# Autodesk Inventor assembly: Pipette Assembly
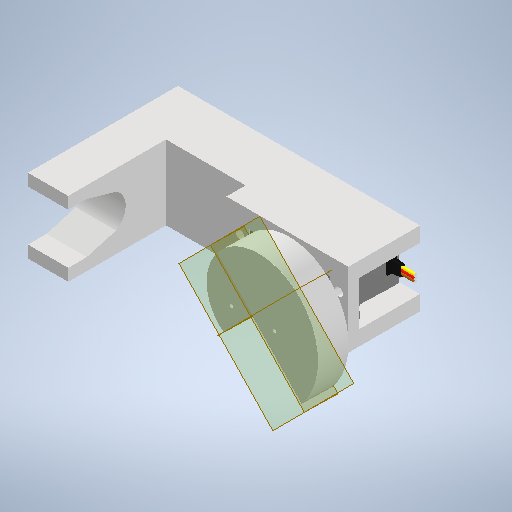
[picture p0: Inventor's stored thumbnail of the model, 512x512]
Saved by Autodesk Inventor 2025.1 (Build 291241000, 241)
## iProperties
Created: 2024-10-19
Part Number: Pipette Assembly
Document SubType Name: Assembly
Designer: 13156
Author: 13156
## Documents named in this file (5)
- C:\Users\13156\Documents\GitHub\Perovskite-Automated-Synthesis-System\CAD\Pipette Assembly.iam
- C:\Users\13156\Downloads\mg996r-servo-3.snapshot.9\mg996R_v2\mg996R_v2\mg996R_v2.ipt
- C:\Users\13156\Desktop\Servo CAD\mg996_arm_2pad\mg996_arm_2pad\mg996_arm_2pad.ipt
- C:\Users\13156\Documents\GitHub\Perovskite-Automated-Synthesis-System\CAD\Holder2.ipt
- C:\Users\13156\Documents\GitHub\Perovskite-Automated-Synthesis-System\CAD\Cam.ipt
## Components (4 placed, 4 different names)
1. mg996R_v2:1 — Mate:1, Insert:1
2. mg996_arm_2pad:1 — Mate:1, Insert:1
3. Holder2:1
4. Cam:1
## Relationships (2: Mate 1, Insert 1)
- Mate:1 (1.5 mm): mg996R_v2:1 ↔ mg996_arm_2pad:1
- Insert:1: mg996R_v2:1 ↔ mg996_arm_2pad:1
